# Autodesk Inventor assembly: side board
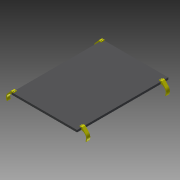
[picture p0: Inventor's stored thumbnail of the model, 180x180]
Saved by Autodesk Inventor 2013 (Build 170138000, 138)
## iProperties
Created: 2013-12-08
Part Number: side board
Document SubType Name: Assembly
Designer: employee
Author: employee
## Documents named in this file (3)
- C:\Users\employee\Desktop\linear simpson 3\side board.iam
- C:\Users\employee\Desktop\linear simpson 3\side board.ipt
- C:\Users\employee\Desktop\linear simpson 3\clip.iam
## Components (5 placed, 2 different names)
1. side board:1 — Mate:1, Mate:2, Mate:3, Mate:4, Mate:5, Mate:6, Mate:7, Mate:8, Flush:1, Flush:2, Flush:3, Flush:4
2. clip:1 [sub-assembly] — Mate:1, Mate:7, Flush:4
3. clip:2 [sub-assembly] — Mate:4, Mate:8, Flush:3
4. clip:3 [sub-assembly] — Mate:3, Mate:5, Flush:2
5. clip:4 [sub-assembly] — Mate:2, Mate:6, Flush:1
## Relationships (12: Mate 8, Flush 4)
- Mate:1: side board:1 ↔ clip:1
- Mate:2: side board:1 ↔ clip:4
- Mate:3: side board:1 ↔ clip:3
- Mate:4: side board:1 ↔ clip:2
- Mate:5: side board:1 ↔ clip:3
- Mate:6: side board:1 ↔ clip:4
- Mate:7: side board:1 ↔ clip:1
- Mate:8: side board:1 ↔ clip:2
- Flush:1: side board:1 ↔ clip:4
- Flush:2: side board:1 ↔ clip:3
- Flush:3 (25 mm): side board:1 ↔ clip:2
- Flush:4 (-25 mm): side board:1 ↔ clip:1
